# Autodesk Inventor assembly: Head
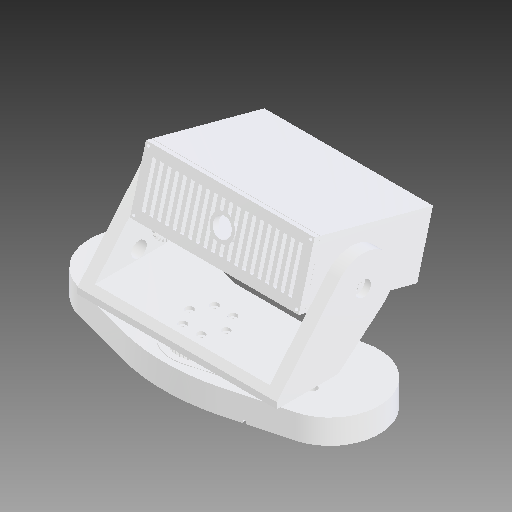
[picture p0: Inventor's stored thumbnail of the model, 512x512]
Saved by Autodesk Inventor 2017 SP1 (Build 210196100, 196)
## iProperties
Created: 2017-06-08
Part Number: Head
Document SubType Name: Assembly
Designer: zallen
Author: zallen
## Documents named in this file (18)
- C:\Users\Zach\Documents\GitHub\tr1\src\Head\Head.iam
- C:\Users\Zach\Documents\GitHub\tr1\src\Head\HA004.ipt
- C:\Users\Zach\Documents\GitHub\tr1\src\Head\HA006.ipt
- C:\Users\Zach\Documents\GitHub\tr1\src\Head\HA007.ipt
- C:\Users\Zach\Documents\GitHub\tr1\lib\DC Motor with Encoder\Motor.ipt
- C:\Users\Zach\Documents\GitHub\tr1\lib\4mm mounting hub.ipt
- C:\Users\Zach\Documents\GitHub\tr1\src\Head\HA009.ipt
- C:\Users\Zach\Documents\GitHub\tr1\lib\Bourns ACE 128\Bourns ACE 128.ipt
- C:\Users\Zach\Documents\GitHub\tr1\src\Head\Head\Design Accelerator\Spur Gears1.iam
- C:\Users\Zach\Documents\Inventor\Content Center Files\R2017\en-US\ISO 7045  H\ISO 7045 - M3 x 16 - 4.8 - H - ISO.ipt
- C:\Users\Zach\Documents\Inventor\Content Center Files\R2017\en-US\ISO 4035(2)\ISO 4035 - M3 - ISO.ipt
- C:\Users\Zach\Documents\GitHub\tr1\src\Body\Arm 2.0 Assembly\AA044.ipt
- C:\Users\Zach\Documents\GitHub\tr1\src\Head\Head\Design Accelerator\Spur Gears2.iam
- C:\Users\Zach\Documents\GitHub\tr1\src\Head\HA013.ipt
- C:\Users\Zach\Documents\GitHub\tr1\src\Head\HA014.ipt
- C:\Users\Zach\Documents\Inventor\Content Center Files\R2017\en-US\ISO 4018\ISO 4018 - M5 x 25.ipt
- C:\Users\Zach\Documents\Inventor\Content Center Files\R2017\en-US\ISO 7045  H\ISO 7045 - M3 x 8 - 4.8 - H - ISO.ipt
- C:\Users\Zach\Documents\GitHub\tr1\lib\Orbbec Astra\Orbbec Astra.iam
## Components (31 placed, 16 different names)
1. HA004:1 — Mate:49, Mate:50, Mate:61, Mate:78, Mate:79, Mate:80, Mate:93, Mate:94, Angle:1, Mate:97, Mate:102, Angle:3, Mate:127, Mate:128, Mate:129, Mate:142, Mate:143, Mate:144
2. HA006:1 — Mate:87, Mate:88, Mate:89
3. HA007:1 — Mate:85, Mate:86, Angle:1, Mate:96, Mate:118, Mate:119, Angle:5, Mate:120, Mate:122, Mate:124, Mate:133, Mate:134, Mate:135, Mate:136, Mate:137
4. HA009:1 — Mate:78, Mate:79, Mate:80, Mate:87, Mate:88, Mate:89, Mate:90, Mate:91, Mate:92, Angle:2, Mate:103, Mate:106, Mate:107, Mate:113, Mate:114, Mate:115, Mate:155, Angle:7, Mate:156, Mate:158, Mate:160
5. Motor:1 — Mate:48, Mate:49, Mate:90
6. Motor:2 — Mate:91, Mate:92
7. 4mm mounting hub:1 — Mate:48, Mate:50
8. 4mm mounting hub:2 — Mate:61, Mate:93, Mate:94, Mate:159
9. 4mm mounting hub:3 — Mate:120, Mate:121, Mate:130, Mate:131, Mate:132
10. Bourns ACE 128:1 — Mate:97, Mate:102, Angle:3, Mate:116, Mate:117, Mate:157
11. Spur Gears:1 [sub-assembly] — Mate:103, Mate:104, Mate:105, Mate:108, Mate:109, Angle:4, Mate:157, Mate:158, Mate:159, Mate:160
12. ISO 7045 H M3 x 16 - 4.8 - H:1 — Mate:104, Mate:105, Mate:110
13. ISO 7045 H M3 x 16 - 4.8 - H:2 — Mate:107, Mate:109, Mate:111
14. ISO 7045 H M3 x 16 - 4.8 - H:3 — Mate:106, Mate:108, Mate:112
15. ISO 4035 M3:1 — Mate:110, Mate:114
16. ISO 4035 M3:2 — Mate:111, Mate:113
17. ISO 4035 M3:3 — Mate:112, Mate:115
18. AA044:1 — Mate:116, Mate:117, Angle:4
19. Bourns ACE 128:2 — Mate:118, Mate:119, Angle:5, Mate:123, Mate:125, Mate:126
20. Spur Gears:2 [sub-assembly] — Mate:121, Mate:122, Mate:123, Mate:124, Angle:6, Mate:127, Mate:128, Mate:129, Mate:130, Mate:131, Mate:132
21. AA044:2 — Mate:125, Mate:126, Angle:6, Mate:153, Mate:154
22. HA013:1 — Mate:133, Mate:134, Mate:135, Mate:136, Mate:137, Mate:138, Mate:139, Mate:140, Mate:141
23. ISO 7045 H M3 x 16 - 4.8 - H:4 — Mate:139, Mate:140
24. ISO 7045 H M3 x 16 - 4.8 - H:5 — Mate:138, Mate:141
25. HA014:1 — Mate:142, Mate:143, Mate:144, Mate:145, Mate:146, Mate:147, Mate:148, Mate:149, Mate:150, Mate:151, Mate:152
26. ISO 4018 M5 x 25:1 — Mate:148, Mate:151
27. ISO 4018 M5 x 25:2 — Mate:147, Mate:152
28. ISO 4018 M5 x 25:3 — Mate:146, Mate:149
29. ISO 4018 M5 x 25:4 — Mate:145, Mate:150
30. ISO 7045 H M3 x 8 - 4.8 - H:1 — Mate:153, Mate:154
31. Orbbec Astra:1 [sub-assembly] — Mate:155, Angle:7, Mate:156
## Relationships (85: Mate 78, Angle 7)
- Mate:48: Motor:1 ↔ 4mm mounting hub:1
- Mate:49: HA004:1 ↔ Motor:1
- Mate:50: HA004:1 ↔ 4mm mounting hub:1
- Mate:61: HA004:1 ↔ 4mm mounting hub:2
- Mate:78: HA004:1 ↔ HA009:1
- Mate:79 (5 mm): HA004:1 ↔ HA009:1
- Mate:80 (5 mm): HA004:1 ↔ HA009:1
- Mate:85: HA007:1
- Mate:86: HA007:1
- Mate:87: HA006:1 ↔ HA009:1
- Mate:88: HA006:1 ↔ HA009:1
- Mate:89: HA006:1 ↔ HA009:1
- Mate:90: HA009:1 ↔ Motor:1
- Mate:91: HA009:1 ↔ Motor:2
- Mate:92: HA009:1 ↔ Motor:2
- Mate:93: HA004:1 ↔ 4mm mounting hub:2
- Mate:94: HA004:1 ↔ 4mm mounting hub:2
- Angle:1 (180 deg): HA004:1 ↔ HA007:1
- Mate:96: HA007:1
- Angle:2 (15 deg): HA009:1
- Mate:97: HA004:1 ↔ Bourns ACE 128:1
- Mate:102: HA004:1 ↔ Bourns ACE 128:1
- Angle:3 (0 deg): HA004:1 ↔ Bourns ACE 128:1
- Mate:103: HA009:1 ↔ Spur Gears:1
- Mate:104: Spur Gears:1 ↔ ISO 7045 H M3 x 16 - 4.8 - H:1
- Mate:105: Spur Gears:1 ↔ ISO 7045 H M3 x 16 - 4.8 - H:1
- Mate:106: HA009:1 ↔ ISO 7045 H M3 x 16 - 4.8 - H:3
- Mate:107: HA009:1 ↔ ISO 7045 H M3 x 16 - 4.8 - H:2
- Mate:108: Spur Gears:1 ↔ ISO 7045 H M3 x 16 - 4.8 - H:3
- Mate:109: Spur Gears:1 ↔ ISO 7045 H M3 x 16 - 4.8 - H:2
- Mate:110: ISO 7045 H M3 x 16 - 4.8 - H:1 ↔ ISO 4035 M3:1
- Mate:111: ISO 7045 H M3 x 16 - 4.8 - H:2 ↔ ISO 4035 M3:2
- Mate:112: ISO 7045 H M3 x 16 - 4.8 - H:3 ↔ ISO 4035 M3:3
- Mate:113: HA009:1 ↔ ISO 4035 M3:2
- Mate:114: HA009:1 ↔ ISO 4035 M3:1
- Mate:115: HA009:1 ↔ ISO 4035 M3:3
- Mate:116: Bourns ACE 128:1 ↔ AA044:1
- Mate:117: Bourns ACE 128:1 ↔ AA044:1
- Angle:4 (0 deg): Spur Gears:1 ↔ AA044:1
- Mate:118: HA007:1 ↔ Bourns ACE 128:2
- Mate:119: HA007:1 ↔ Bourns ACE 128:2
- Angle:5 (0 deg): HA007:1 ↔ Bourns ACE 128:2
- Mate:120: HA007:1 ↔ 4mm mounting hub:3
- Mate:121: 4mm mounting hub:3 ↔ Spur Gears:2
- Mate:122: HA007:1 ↔ Spur Gears:2
- Mate:123: Bourns ACE 128:2 ↔ Spur Gears:2
- Mate:124: HA007:1 ↔ Spur Gears:2
- Mate:125: Bourns ACE 128:2 ↔ AA044:2
- Mate:126: Bourns ACE 128:2 ↔ AA044:2
- Angle:6 (0 deg): Spur Gears:2 ↔ AA044:2
- Mate:127: HA004:1 ↔ Spur Gears:2
- Mate:128: HA004:1 ↔ Spur Gears:2
- Mate:129: HA004:1 ↔ Spur Gears:2
- Mate:130: 4mm mounting hub:3 ↔ Spur Gears:2
- Mate:131: 4mm mounting hub:3 ↔ Spur Gears:2
- Mate:132: 4mm mounting hub:3 ↔ Spur Gears:2
- Mate:133: HA007:1 ↔ HA013:1
- Mate:134: HA007:1 ↔ HA013:1
- Mate:135: HA007:1 ↔ HA013:1
- Mate:136: HA007:1 ↔ HA013:1
- Mate:137: HA007:1 ↔ HA013:1
- Mate:138: HA013:1 ↔ ISO 7045 H M3 x 16 - 4.8 - H:5
- Mate:139: HA013:1 ↔ ISO 7045 H M3 x 16 - 4.8 - H:4
- Mate:140: HA013:1 ↔ ISO 7045 H M3 x 16 - 4.8 - H:4
- Mate:141: HA013:1 ↔ ISO 7045 H M3 x 16 - 4.8 - H:5
- Mate:142: HA004:1 ↔ HA014:1
- Mate:143: HA004:1 ↔ HA014:1
- Mate:144: HA004:1 ↔ HA014:1
- Mate:145: HA014:1 ↔ ISO 4018 M5 x 25:4
- Mate:146: HA014:1 ↔ ISO 4018 M5 x 25:3
- Mate:147: HA014:1 ↔ ISO 4018 M5 x 25:2
- Mate:148: HA014:1 ↔ ISO 4018 M5 x 25:1
- Mate:149: HA014:1 ↔ ISO 4018 M5 x 25:3
- Mate:150: HA014:1 ↔ ISO 4018 M5 x 25:4
- Mate:151: HA014:1 ↔ ISO 4018 M5 x 25:1
- Mate:152: HA014:1 ↔ ISO 4018 M5 x 25:2
- Mate:153: AA044:2 ↔ ISO 7045 H M3 x 8 - 4.8 - H:1
- Mate:154: AA044:2 ↔ ISO 7045 H M3 x 8 - 4.8 - H:1
- Mate:155: HA009:1 ↔ Orbbec Astra:1
- Angle:7 (180 deg): HA009:1 ↔ Orbbec Astra:1
- Mate:156: HA009:1 ↔ Orbbec Astra:1
- Mate:157: Bourns ACE 128:1 ↔ Spur Gears:1
- Mate:158: HA009:1 ↔ Spur Gears:1
- Mate:159: 4mm mounting hub:2 ↔ Spur Gears:1
- Mate:160: HA009:1 ↔ Spur Gears:1
